# Autodesk Inventor assembly: A2017_T5_02
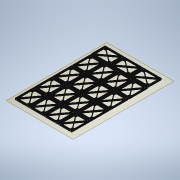
[picture p0: Inventor's stored thumbnail of the model, 180x180]
Saved by Autodesk Inventor 2022 (Build 260153000, 153)
## iProperties
Created: 2022-09-28
Part Number: A2017_T5_02
Document SubType Name: Assembly
Designer: Masato
Author: Masato
## Documents named in this file (3)
- C:\Users\ヨコオリク\Documents\CITBrains\SUSTAINA-OP\Cam\A2017_T5\A2017_T5_02.iam
- C:\Users\ヨコオリク\Documents\CITBrains\SUSTAINA-OP\Cam\DisposableBoard.ipt
- C:\Users\ヨコオリク\Documents\CITBrains\SUSTAINA-OP\LowerBody\Link\FrontLink_diagonal.ipt
## Components (20 placed, 2 different names)
1. DisposableBoard:1 — フラッシュ:1, フラッシュ:2, フラッシュ:3, フラッシュ:4, フラッシュ:5, フラッシュ:6, フラッシュ:8, フラッシュ:9
2. FrontLink_diagonal:1 — メイト:1, フラッシュ:5, フラッシュ:6
3. FrontLink_diagonal:2
4. FrontLink_diagonal:3
5. FrontLink_diagonal:4
6. FrontLink_diagonal:5
7. FrontLink_diagonal:6
8. FrontLink_diagonal:7
9. FrontLink_diagonal:8
10. FrontLink_diagonal:9
11. FrontLink_diagonal:10
12. FrontLink_diagonal:11
13. FrontLink_diagonal:12
14. FrontLink_diagonal:13 — メイト:3
15. FrontLink_diagonal:14
16. FrontLink_diagonal:15
17. FrontLink_diagonal:16
18. FrontLink_diagonal:17 — フラッシュ:8, メイト:3, フラッシュ:9
19. FrontLink_diagonal:18
20. FrontLink_diagonal:19
## Component patterns: (16 elements, first: FrontLink_diagonal:1), (3 elements, first: FrontLink_diagonal:17)
## Relationships (10: Flush 8, Mate 2)
- フラッシュ:1 [Flush]: DisposableBoard:1
- フラッシュ:2 [Flush]: DisposableBoard:1
- フラッシュ:3 [Flush]: DisposableBoard:1
- フラッシュ:4 [Flush]: DisposableBoard:1
- メイト:1 [Mate]: FrontLink_diagonal:1
- フラッシュ:5 [Flush] (2 mm): DisposableBoard:1 ↔ FrontLink_diagonal:1
- フラッシュ:6 [Flush] (2 mm): DisposableBoard:1 ↔ FrontLink_diagonal:1
- フラッシュ:8 [Flush] (2 mm): DisposableBoard:1 ↔ FrontLink_diagonal:17
- メイト:3 [Mate] (2.1 mm): FrontLink_diagonal:13 ↔ FrontLink_diagonal:17
- フラッシュ:9 [Flush] (2 mm): DisposableBoard:1 ↔ FrontLink_diagonal:17
